# Autodesk Inventor assembly: first_floor2
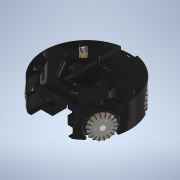
[picture p0: Inventor's stored thumbnail of the model, 180x180]
Saved by Autodesk Inventor 2020.4 (Build 244396000, 396)
## iProperties
Created: 2021-05-09
Part Number: first_floor2
Document SubType Name: Assembly
Designer: Acer
Author: Acer
## Documents named in this file (3)
- C:\Users\Acer\Documents\MATLAB\Doutorado\CAD\Inventor\first_floor\first_floor2.iam
- C:\Users\Acer\Documents\MATLAB\Doutorado\CAD\Inventor\first_floor\Base_RoboCIn.ipt
- C:\Users\Acer\Documents\MATLAB\Doutorado\CAD\Inventor\first_floor\Wheel\RoboCinWheel.iam
## Components (5 placed, 2 different names)
1. Base_RoboCIn:1 — Mate:28, Mate:29, Mate:30, Mate:31, Mate:32, Mate:33, Mate:34, Mate:35
2. RoboCinWheel:1 [sub-assembly] — Mate:28, Mate:29
3. RoboCinWheel:2 [sub-assembly] — Mate:30, Mate:31
4. RoboCinWheel:3 [sub-assembly] — Mate:34, Mate:35
5. RoboCinWheel:4 [sub-assembly] — Mate:32, Mate:33
## Relationships (8: Mate 8)
- Mate:28: Base_RoboCIn:1 ↔ RoboCinWheel:1
- Mate:29 (1 mm): Base_RoboCIn:1 ↔ RoboCinWheel:1
- Mate:30: Base_RoboCIn:1 ↔ RoboCinWheel:2
- Mate:31 (1 mm): Base_RoboCIn:1 ↔ RoboCinWheel:2
- Mate:32: Base_RoboCIn:1 ↔ RoboCinWheel:4
- Mate:33 (1 mm): Base_RoboCIn:1 ↔ RoboCinWheel:4
- Mate:34: Base_RoboCIn:1 ↔ RoboCinWheel:3
- Mate:35 (1 mm): Base_RoboCIn:1 ↔ RoboCinWheel:3
